# Autodesk Inventor assembly: DribblerUnit
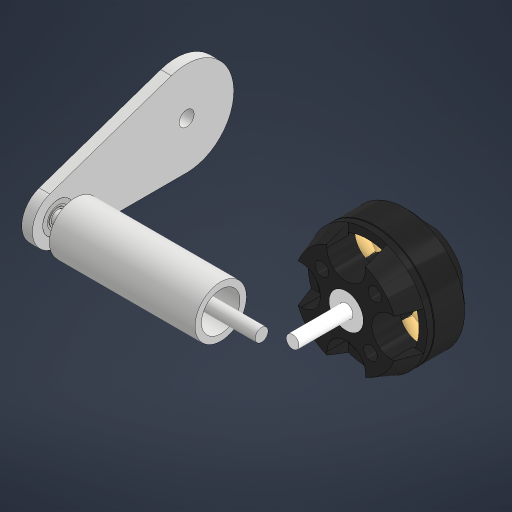
[picture p0: Inventor's stored thumbnail of the model, 512x512]
Saved by Autodesk Inventor 2024.2 (Build 282272000, 272)
## iProperties
Created: 2023-12-27
Part Number: DribblerUnit
Document SubType Name: Assembly
Designer: Hanaoka
Author: Hanaoka
## Documents named in this file (6)
- G:\共有ドライブ\reRo\05_個人\hanaoka\inventor\DribblerUnit\DribblerUnit.iam
- G:\共有ドライブ\reRo\05_個人\hanaoka\inventor\DribblerUnit\C2822_BLDC.ipt
- G:\共有ドライブ\reRo\05_個人\hanaoka\inventor\DribblerUnit\Shaft_D3.ipt
- G:\共有ドライブ\reRo\05_個人\hanaoka\inventor\DribblerUnit\tube.ipt
- G:\共有ドライブ\reRo\05_個人\hanaoka\inventor\DribblerUnit\Bearing_C-FL673ZZ.ipt
- G:\共有ドライブ\reRo\05_個人\hanaoka\inventor\DribblerUnit\Main_Frame.ipt
## Components (5 placed, 5 different names)
1. C2822_BLDC:1
2. Shaft_D3:1 — 挿入:2
3. tube:1
4. Bearing_C-FL673ZZ:1 — 挿入:1, 挿入:2
5. Main_Frame:1 — 挿入:1
## Relationships (2: Insert 2)
- 挿入:1 [Insert]: Bearing_C-FL673ZZ:1 ↔ Main_Frame:1
- 挿入:2 [Insert]: Shaft_D3:1 ↔ Bearing_C-FL673ZZ:1
